# Autodesk Inventor assembly: 12x12x3.758324274 in
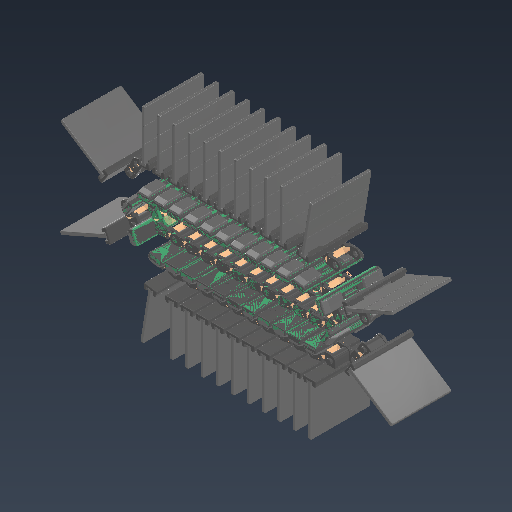
[picture p0: Inventor's stored thumbnail of the model, 512x512]
Saved by Autodesk Inventor 2021 (Build 250183000, 183)
## iProperties
RuleStatus: InUse
Created: 2020-07-07
Part Number: 12x12x3.758324274 in
Document SubType Name: Assembly
Designer: yuany
AfterDocOpen0: Open Form
Author: yuany
## Documents named in this file (9)
- C:\Users\Robotics\Desktop\CAD\Library 1.2\Motion\Chain + Tank Tread\Parametric\Generated\12x12x3.758324274 in.iam
- C:\Users\Robotics\Desktop\CAD\Library 1.2\Motion\Chain + Tank Tread\Parametric\Workpoint Pattern.ipt
- C:\Users\Robotics\Desktop\CAD\Library 1.2\Motion\Chain + Tank Tread\High Strength Chain Link.ipt
- C:\Users\Robotics\Desktop\CAD\Library 1.2\Motion\Chain + Tank Tread\Tank Tread Traction Link.ipt
- C:\Users\Robotics\Desktop\CAD\Library 1.2\Motion\Chain + Tank Tread\Tread Link.ipt
- C:\Users\Robotics\Desktop\CAD\Library 1.2\Motion\Chain + Tank Tread\Chain Attachment Link.ipt
- C:\Users\Robotics\Desktop\CAD\Library 1.2\Motion\Chain + Tank Tread\Short Flap.ipt
- C:\Users\Robotics\Desktop\CAD\Library 1.2\Motion\Chain + Tank Tread\Medium Flap.ipt
- C:\Users\Robotics\Desktop\CAD\Library 1.2\Motion\Chain + Tank Tread\Tall Flap.ipt
## Components (183 placed, 8 different names)
1. Workpoint Pattern:3 — Mate:1, Mate:2, Mate:3
2. High Strength Chain Link:1 — Mate:1, Mate:2, Mate:3, Flush:1, Mate:4, Angle:1
3. High Strength Chain Link:2
4. High Strength Chain Link:3
5. High Strength Chain Link:4
6. High Strength Chain Link:5
7. High Strength Chain Link:6
8. High Strength Chain Link:7
9. High Strength Chain Link:8
10. High Strength Chain Link:9
11. High Strength Chain Link:10
12. High Strength Chain Link:11
13. High Strength Chain Link:12
14. High Strength Chain Link:13
15. High Strength Chain Link:14
16. High Strength Chain Link:15
17. High Strength Chain Link:16
18. High Strength Chain Link:17
19. High Strength Chain Link:18
20. High Strength Chain Link:19
21. High Strength Chain Link:20
22. High Strength Chain Link:21
23. High Strength Chain Link:22
24. High Strength Chain Link:23
25. High Strength Chain Link:24
26. High Strength Chain Link:25
27. High Strength Chain Link:26
28. Tank Tread Traction Link:1 — Flush:1, Mate:4, Angle:1, Flush:2, Mate:5, Angle:2
29. Tank Tread Traction Link:2
30. Tank Tread Traction Link:3
31. Tank Tread Traction Link:4
32. Tank Tread Traction Link:5
33. Tank Tread Traction Link:6
34. Tank Tread Traction Link:7
35. Tank Tread Traction Link:8
36. Tank Tread Traction Link:9
37. Tank Tread Traction Link:10
38. Tank Tread Traction Link:11
39. Tank Tread Traction Link:12
40. Tank Tread Traction Link:13
41. Tank Tread Traction Link:14
42. Tank Tread Traction Link:15
43. Tank Tread Traction Link:16
44. Tank Tread Traction Link:17
45. Tank Tread Traction Link:18
46. Tank Tread Traction Link:19
47. Tank Tread Traction Link:20
48. Tank Tread Traction Link:21
49. Tank Tread Traction Link:22
50. Tank Tread Traction Link:23
51. Tank Tread Traction Link:24
52. Tank Tread Traction Link:25
53. Tank Tread Traction Link:26
54. Tread Link:1 — Flush:2, Mate:5, Angle:2, Flush:3, Mate:6, Angle:3
55. Tread Link:2
56. Tread Link:3
57. Tread Link:4
58. Tread Link:5
59. Tread Link:6
60. Tread Link:7
61. Tread Link:8
62. Tread Link:9
63. Tread Link:10
64. Tread Link:11
65. Tread Link:12
66. Tread Link:13
67. Tread Link:14
68. Tread Link:15
69. Tread Link:16
70. Tread Link:17
71. Tread Link:18
72. Tread Link:19
73. Tread Link:20
74. Tread Link:21
75. Tread Link:22
76. Tread Link:23
77. Tread Link:24
78. Tread Link:25
79. Tread Link:26
80. Chain Attachment Link:1 — Flush:3, Mate:6, Angle:3
81. Chain Attachment Link:2
82. Chain Attachment Link:3
83. Chain Attachment Link:4
84. Chain Attachment Link:5
85. Chain Attachment Link:6
86. Chain Attachment Link:7
87. Chain Attachment Link:8
88. Chain Attachment Link:9
89. Chain Attachment Link:10
90. Chain Attachment Link:11
91. Chain Attachment Link:12
92. Chain Attachment Link:13
93. Chain Attachment Link:14
94. Chain Attachment Link:15
95. Chain Attachment Link:16
96. Chain Attachment Link:17
97. Chain Attachment Link:18
98. Chain Attachment Link:19
99. Chain Attachment Link:20
100. Chain Attachment Link:21
101. Chain Attachment Link:22
102. Chain Attachment Link:23
103. Chain Attachment Link:24
104. Chain Attachment Link:25
105. Chain Attachment Link:26
106. Short Flap:1 [sub-assembly]
107. Short Flap:2 [sub-assembly]
108. Short Flap:3 [sub-assembly]
109. Short Flap:4 [sub-assembly]
110. Short Flap:5 [sub-assembly]
111. Short Flap:6 [sub-assembly]
112. Short Flap:7 [sub-assembly]
113. Short Flap:8 [sub-assembly]
114. Short Flap:9 [sub-assembly]
115. Short Flap:10 [sub-assembly]
116. Short Flap:11 [sub-assembly]
117. Short Flap:12 [sub-assembly]
118. Short Flap:13 [sub-assembly]
119. Short Flap:14 [sub-assembly]
120. Short Flap:15 [sub-assembly]
121. Short Flap:16 [sub-assembly]
122. Short Flap:17 [sub-assembly]
123. Short Flap:18 [sub-assembly]
124. Short Flap:19 [sub-assembly]
125. Short Flap:20 [sub-assembly]
126. Short Flap:21 [sub-assembly]
127. Short Flap:22 [sub-assembly]
128. Short Flap:23 [sub-assembly]
129. Short Flap:24 [sub-assembly]
130. Short Flap:25 [sub-assembly]
131. Short Flap:26 [sub-assembly]
132. Medium Flap:1 [sub-assembly]
133. Medium Flap:2 [sub-assembly]
134. Medium Flap:3 [sub-assembly]
135. Medium Flap:4 [sub-assembly]
136. Medium Flap:5 [sub-assembly]
137. Medium Flap:6 [sub-assembly]
138. Medium Flap:7 [sub-assembly]
139. Medium Flap:8 [sub-assembly]
140. Medium Flap:9 [sub-assembly]
141. Medium Flap:10 [sub-assembly]
142. Medium Flap:11 [sub-assembly]
143. Medium Flap:12 [sub-assembly]
144. Medium Flap:13 [sub-assembly]
145. Medium Flap:14 [sub-assembly]
146. Medium Flap:15 [sub-assembly]
147. Medium Flap:16 [sub-assembly]
148. Medium Flap:17 [sub-assembly]
149. Medium Flap:18 [sub-assembly]
150. Medium Flap:19 [sub-assembly]
151. Medium Flap:20 [sub-assembly]
152. Medium Flap:21 [sub-assembly]
153. Medium Flap:22 [sub-assembly]
154. Medium Flap:23 [sub-assembly]
155. Medium Flap:24 [sub-assembly]
156. Medium Flap:25 [sub-assembly]
157. Medium Flap:26 [sub-assembly]
158. Tall Flap:1 [sub-assembly]
159. Tall Flap:2 [sub-assembly]
160. Tall Flap:3 [sub-assembly]
161. Tall Flap:4 [sub-assembly]
162. Tall Flap:5 [sub-assembly]
163. Tall Flap:6 [sub-assembly]
164. Tall Flap:7 [sub-assembly]
165. Tall Flap:8 [sub-assembly]
166. Tall Flap:9 [sub-assembly]
167. Tall Flap:10 [sub-assembly]
168. Tall Flap:11 [sub-assembly]
169. Tall Flap:12 [sub-assembly]
170. Tall Flap:13 [sub-assembly]
171. Tall Flap:14 [sub-assembly]
172. Tall Flap:15 [sub-assembly]
173. Tall Flap:16 [sub-assembly]
174. Tall Flap:17 [sub-assembly]
175. Tall Flap:18 [sub-assembly]
176. Tall Flap:19 [sub-assembly]
177. Tall Flap:20 [sub-assembly]
178. Tall Flap:21 [sub-assembly]
179. Tall Flap:22 [sub-assembly]
180. Tall Flap:23 [sub-assembly]
181. Tall Flap:24 [sub-assembly]
182. Tall Flap:25 [sub-assembly]
183. Tall Flap:26 [sub-assembly]
## Component patterns: Chain (26 elements), Traction (26 elements), Tread (26 elements), Chain Attachment (26 elements), Short Flaps (26 elements), Medium Flaps (26 elements), Tall Flaps (26 elements)
## Relationships (12: Mate 6, Flush 3, Angle 3)
- Mate:1: Workpoint Pattern:3 ↔ High Strength Chain Link:1
- Mate:2 (11.938 mm): Workpoint Pattern:3 ↔ High Strength Chain Link:1
- Mate:3: Workpoint Pattern:3 ↔ High Strength Chain Link:1
- Flush:1: High Strength Chain Link:1 ↔ Tank Tread Traction Link:1
- Mate:4: High Strength Chain Link:1 ↔ Tank Tread Traction Link:1
- Angle:1 (180 deg): High Strength Chain Link:1 ↔ Tank Tread Traction Link:1
- Flush:2: Tank Tread Traction Link:1 ↔ Tread Link:1
- Mate:5: Tank Tread Traction Link:1 ↔ Tread Link:1
- Angle:2 (0 deg): Tank Tread Traction Link:1 ↔ Tread Link:1
- Flush:3: Tread Link:1 ↔ Chain Attachment Link:1
- Mate:6: Tread Link:1 ↔ Chain Attachment Link:1
- Angle:3 (0 deg): Tread Link:1 ↔ Chain Attachment Link:1
## Named parameters: Center_Distance = 95.46144 mm, Sprocket1 = 19.558 mm, Sprocket2 = 19.558 mm, CenterDistance = 95.46144 mm, d5_1 = 95.46144 mm, d6_1 = 95.46144 mm, d7_1 = 30.72163 mm, d8_1 = 30.72163 mm
